# Autodesk Inventor assembly: GuiasHGH30HA2T1050Z0H_FILE_1
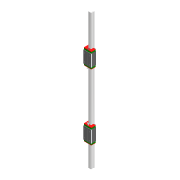
[picture p0: Inventor's stored thumbnail of the model, 180x180]
Saved by Autodesk Inventor 2021 (Build 250183000, 183)
## iProperties
Company: CADClick - www.CADClick.com
Created: 2021-08-23
Part Number: GuiasHGH30HA2T1050Z0H_FILE_1
Description: STEP AP214
Document SubType Name: Assembly
Designer: Santiago Suárez
Authority: unknown authorization
Title: cctmp_2626557F-3D31-4675-BB22-368ADEDF7ABC_2021_08_23_02_05_21_0438..stp
Author: HIWIN GmbH
Revision Number: NONE
Preprocessor: Spatial InterOp 3D
## Documents named in this file (4)
- C:\Users\Santiago Suárez\Documents\GitHub\Dis.-Mecatronico-E6\inventor proyecto\Guias\GuiasHGH30HA2T1050Z0H_FILE_1.iam
- C:\Users\Santiago Suárez\Documents\GitHub\Dis.-Mecatronico-E6\inventor proyecto\Guias\GuiasHGH30HA2T1050Z0H_FILE_2.ipt
- C:\Users\Santiago Suárez\Documents\GitHub\Dis.-Mecatronico-E6\inventor proyecto\Guias\GuiasHGH30HA2T1050Z0H_FILE_1.ipt
- C:\Users\Santiago Suárez\Documents\GitHub\Dis.-Mecatronico-E6\inventor proyecto\Guias\GuiasHGH30HA2T1050Z0H_FILE.ipt
## Components (3 placed, 3 different names)
1. GuiasHGH30HA2T1050Z0H_FILE_2 — Slider:2
2. GuiasHGH30HA2T1050Z0H_FILE_1 — Slider:1
3. GuiasHGH30HA2T1050Z0H_FILE — Slider:1, Slider:2
## Relationships (2: TranslationJoint 2)
- Slider:1 [TranslationJoint]: GuiasHGH30HA2T1050Z0H_FILE_1 ↔ GuiasHGH30HA2T1050Z0H_FILE
- Slider:2 [TranslationJoint]: GuiasHGH30HA2T1050Z0H_FILE_2 ↔ GuiasHGH30HA2T1050Z0H_FILE
